# Autodesk Inventor assembly: s-assy-scara-magnet
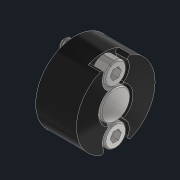
[picture p0: Inventor's stored thumbnail of the model, 180x180]
Saved by Autodesk Inventor 2022 (Build 260153000, 153)
## iProperties
Created: 2021-07-15
Part Number: s-assy-scara-magnet
Document SubType Name: Assembly
Designer: yuta0
Author: yuta0
## Documents named in this file (4)
- C:\Users\yuta0\Documents\GitHub\catchrobo_hardware\assy-scara\s-assy-scara-magnet.iam
- C:\Users\yuta0\Documents\GitHub\catchrobo_hardware\assy-robot\magnet.ipt
- C:\Users\yuta0\Documents\GitHub\catchrobo_hardware\assy-scara\scara-base21.ipt
- C:\Users\yuta0\Documents\GitHub\catchrobo_hardware\assy-scara\CB2_5-8.ipt
## Components (4 placed, 3 different names)
1. scara-base21:1 — メイト:1, メイト:2, メイト:3, メイト:4
2. magnet:1 — メイト:1, メイト:2
3. CB2_5-8:1 — メイト:3, メイト:4
4. CB2_5-8:2
## Component patterns: (2 elements, first: CB2_5-8:1)
## Relationships (4: Mate 4)
- メイト:1 [Mate]: scara-base21:1 ↔ magnet:1
- メイト:2 [Mate]: scara-base21:1 ↔ magnet:1
- メイト:3 [Mate]: scara-base21:1 ↔ CB2_5-8:1
- メイト:4 [Mate]: scara-base21:1 ↔ CB2_5-8:1
